# Autodesk Inventor assembly: xtion_custom_assembly
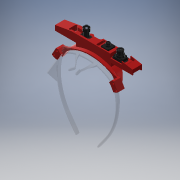
[picture p0: Inventor's stored thumbnail of the model, 180x180]
Saved by Autodesk Inventor 2017 (Build 210142000, 142)
## iProperties
Created: 2016-11-18
Part Number: xtion_custom_assembly
Document SubType Name: Assembly
Designer: Ali
Author: Ali
## Documents named in this file (9)
- C:\Users\Alistair\Dropbox\Work\HeadSLAM\prototype-1\xtion_custom_assembly.iam
- C:\Users\Alistair\Dropbox\Work\HeadSLAM\xtion-internal\xtion_heatsink.ipt
- C:\Users\Alistair\Dropbox\Work\HeadSLAM\xtion-internal\xtion_projector.ipt
- C:\Users\Alistair\Dropbox\Work\HeadSLAM\xtion-internal\xtion_rgb_cam.ipt
- C:\Users\Alistair\Dropbox\Work\HeadSLAM\xtion-internal\xtion_ir_cam.ipt
- C:\Users\Alistair\Dropbox\Work\HeadSLAM\prototype-1\xtion_custom.ipt
- C:\Users\Alistair\Dropbox\Work\HeadSLAM\xtion-internal\xtion_mainboard.ipt
- C:\Users\Alistair\Dropbox\Work\HeadSLAM\pupil\pupil_frame_full.ipt
- C:\Users\Alistair\Dropbox\Work\HeadSLAM\prototype-1\mounting.ipt
## Components (8 placed, 8 different names)
1. xtion_heatsink:1
2. xtion_projector:1
3. xtion_rgb_cam:1
4. xtion_ir_cam:1
5. xtion_custom:1 — Flush:1, Rigid:4
6. pupil_frame_full:1
7. xtion_mainboard:1 — Rigid:4
8. mounting:1
## Relationships (2: Flush 1, WeldJoint 1)
- Flush:1: xtion_custom:1
- Rigid:4 [WeldJoint]: xtion_custom:1 ↔ xtion_mainboard:1
